# Autodesk Inventor assembly: CY8CKIT-059
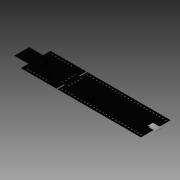
[picture p0: Inventor's stored thumbnail of the model, 180x180]
Saved by Autodesk Inventor 2016 SP1 (Build 200210100, 210)
## iProperties
Category: Control System
Company: Autodesk Inc.
Created: 2015-11-22
Part Number: CY8CKIT-059
Document SubType Name: Assembly
Designer: Autodesk Inc.
Catalog Web Link: http://www.cypress.com/documentation/development-kitsboards/cy8ckit-059-psoc-5lp-prototyping-kit
Vendor: Cypress
Author: Autodesk Inc.
## Documents named in this file (3)
- D:\FIRST\FRC KOP 2016\FRC KOP 2016\Control System\fc16-030_ProtoKit.iam
- D:\FIRST\FRC KOP 2016\FRC FIRSTChoice 2016\Parts\fr16-030_ProtoKit.ipt
- D:\FIRST\FRC KOP 2016\FRC KOP 2016\Control System\Parts\fc16-030_USB_PCB.ipt
## Components (2 placed, 2 different names)
1. fr16-030_ProtoKit:1 — Mate:1, Flush:1, Mate:3, Angle:2
2. fc16-030_USB_PCB:1 — Mate:1, Flush:1, Mate:2, Angle:1
## Relationships (7: Mate 4, Angle 2, Flush 1)
- Mate:1: fr16-030_ProtoKit:1 ↔ fc16-030_USB_PCB:1
- Flush:1 (-2 mm): fr16-030_ProtoKit:1 ↔ fc16-030_USB_PCB:1
- Mate:2: fc16-030_USB_PCB:1
- Angle:1 (0 deg): fc16-030_USB_PCB:1
- Mate:3: fr16-030_ProtoKit:1
- Angle:2 (0 deg): fr16-030_ProtoKit:1
- Mate:4
